# Autodesk Inventor assembly: highlevel
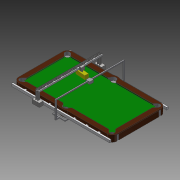
[picture p0: Inventor's stored thumbnail of the model, 180x180]
Saved by Autodesk Inventor 2015 (Build 190159000, 159)
## iProperties
Created: 2016-12-01
Part Number: highlevel
Document SubType Name: Assembly
Designer: Ernest
Author: Ernest
## Documents named in this file (11)
- C:\Users\Guy\Documents\Fourth Year\Capstone\git\Capstone-Project\doc\CAD\HighLevel\highlevel.iam
- C:\Users\Guy\Documents\Fourth Year\Capstone\git\Capstone-Project\doc\CAD\Pool Table\Table_Model.ipt
- C:\Users\Guy\Documents\Fourth Year\Capstone\git\Capstone-Project\doc\CAD\HighLevel\Rail.ipt
- C:\Users\Guy\Documents\Fourth Year\Capstone\git\Capstone-Project\doc\CAD\HighLevel\ArmBase3.ipt
- C:\Users\Guy\Documents\Fourth Year\Capstone\git\Capstone-Project\doc\CAD\HighLevel\Arm.ipt
- C:\Users\Guy\Documents\Fourth Year\Capstone\git\Capstone-Project\doc\CAD\HighLevel\Bridge.ipt
- C:\Users\Guy\Documents\Fourth Year\Capstone\git\Capstone-Project\doc\CAD\HighLevel\YRail.ipt
- C:\Users\Guy\Documents\Fourth Year\Capstone\git\Capstone-Project\doc\CAD\HighLevel\EF-Base.ipt
- C:\Users\Guy\Documents\Fourth Year\Capstone\git\Capstone-Project\doc\CAD\HighLevel\EF-Arm.ipt
- C:\Users\Guy\Documents\Fourth Year\Capstone\git\Capstone-Project\doc\CAD\HighLevel\End-Effector.ipt
- C:\Users\Guy\Documents\Fourth Year\Capstone\git\Capstone-Project\doc\CAD\HighLevel\CameraMount.ipt
## Components (13 placed, 10 different names)
1. Table_Model:1 — Mate:1, Flush:1, Mate:2, Flush:4, Mate:12, Flush:21, Mate:13
2. Rail:1 — Mate:1, Flush:1, Flush:2, Flush:3, Flush:4, Mate:4, Flush:20
3. Rail:2 — Flush:2, Flush:3, Mate:2, Mate:3
4. ArmBase3:1 — Flush:5, Flush:6, Mate:4, Mate:5, Flush:10, Flush:12, Flush:20
5. ArmBase3:2 — Flush:5, Flush:6, Mate:3, Flush:11
6. Arm:1 — Flush:8, Flush:9, Mate:5, Flush:10, Flush:12
7. Arm:2 — Flush:8, Flush:9, Flush:11, Mate:6, Flush:13, Flush:14
8. Bridge:1 — Mate:6, Flush:13, Flush:14, Mate:7, Flush:15, Flush:16
9. YRail:1 — Mate:7, Flush:15, Flush:16, Mate:8, Flush:17
10. EF-Base:1 — Mate:8, Flush:17, Mate:9, Flush:18, Flush:19
11. EF-Arm:1 — Mate:9, Mate:10, Mate:11, Flush:18, Flush:19
12. End-Effector:1 — Mate:10, Mate:11
13. CameraMount:1 — Mate:12, Flush:21, Mate:13
## Relationships (33: Flush 20, Mate 13)
- Mate:1: Table_Model:1 ↔ Rail:1
- Flush:1: Table_Model:1 ↔ Rail:1
- Flush:2: Rail:1 ↔ Rail:2
- Flush:3: Rail:1 ↔ Rail:2
- Mate:2: Table_Model:1 ↔ Rail:2
- Flush:4 (42.261 mm): Table_Model:1 ↔ Rail:1
- Flush:5: ArmBase3:1 ↔ ArmBase3:2
- Flush:6: ArmBase3:1 ↔ ArmBase3:2
- Mate:3: Rail:2 ↔ ArmBase3:2
- Mate:4: Rail:1 ↔ ArmBase3:1
- Flush:8: Arm:1 ↔ Arm:2
- Flush:9: Arm:1 ↔ Arm:2
- Mate:5: ArmBase3:1 ↔ Arm:1
- Flush:10 (20 mm): ArmBase3:1 ↔ Arm:1
- Flush:11 (20 mm): ArmBase3:2 ↔ Arm:2
- Flush:12 (58 mm): ArmBase3:1 ↔ Arm:1
- Mate:6: Arm:2 ↔ Bridge:1
- Flush:13: Arm:2 ↔ Bridge:1
- Flush:14: Arm:2 ↔ Bridge:1
- Mate:7: Bridge:1 ↔ YRail:1
- Flush:15: Bridge:1 ↔ YRail:1
- Flush:16 (10 mm): Bridge:1 ↔ YRail:1
- Mate:8: YRail:1 ↔ EF-Base:1
- Flush:17 (-17 mm): YRail:1 ↔ EF-Base:1
- Mate:9: EF-Base:1 ↔ EF-Arm:1
- Mate:10: EF-Arm:1 ↔ End-Effector:1
- Mate:11: EF-Arm:1 ↔ End-Effector:1
- Flush:18 (11.432 mm): EF-Base:1 ↔ EF-Arm:1
- Flush:19 (29.836 mm): EF-Base:1 ↔ EF-Arm:1
- Flush:20 (-15 mm): Rail:1 ↔ ArmBase3:1
- Mate:12: Table_Model:1 ↔ CameraMount:1
- Flush:21: Table_Model:1 ↔ CameraMount:1
- Mate:13 (1035.5 mm): Table_Model:1 ↔ CameraMount:1
